# Autodesk Inventor assembly: A-00-0
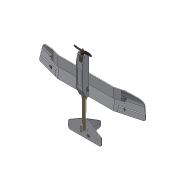
[picture p0: Inventor's stored thumbnail of the model, 180x180]
Saved by Autodesk Inventor 2019 (Build 230136000, 136)
## iProperties
Created: 2022-04-09
Part Number: A-00-0
Document SubType Name: Assembly
Designer: solyo
Mass: 180.895 g
Surface Area: 4249.9 cm^2
Volume: 1031.43 cm^3
Density: 0.175382 g/cm^3
Author: solyo
## Documents named in this file (5)
- D:\Modelling\RC\RC Trainer V1\ASSEMBLY\A-00-0-MAIN\A-00-0.iam
- D:\Modelling\RC\RC Trainer V1\ASSEMBLY\A-02-0-WING\A-02-0.iam
- D:\Modelling\RC\RC Trainer V1\ASSEMBLY\A-01-0-FUSELAGE\A-01-0.iam
- D:\Modelling\RC\RC Trainer V1\Parts\C-00-0-BATTERY_600MAH\C-00-0.ipt
- D:\Modelling\RC\RC Trainer V1\PARTS\C-06-0-5030_PROPELLER\C-06-0.ipt
## Components (4 placed, 4 different names)
1. A-02-0:1 [sub-assembly]
2. A-01-0:1 [sub-assembly] — Flush:18, Mate:44, Mate:45, Insert:1
3. C-00-0:1 — Flush:17, Mate:44, Mate:45
4. C-06-0:1 — Insert:1
## Relationships (11: Flush 7, Mate 3, Insert 1)
- [Flush]: A-01-0:1
- [Flush]: A-01-0:1
- [Flush]: A-01-0:1
- [Flush]: A-02-0:1 ↔ A-01-0:1
- [Flush]: A-02-0:1 ↔ A-01-0:1
- [Mate]: A-02-0:1 ↔ A-01-0:1
- Flush:17: C-00-0:1
- Flush:18: A-01-0:1
- Mate:44: A-01-0:1 ↔ C-00-0:1
- Mate:45: A-01-0:1 ↔ C-00-0:1
- Insert:1: A-01-0:1 ↔ C-06-0:1
